# Autodesk Inventor assembly: Tele
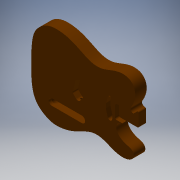
[picture p0: Inventor's stored thumbnail of the model, 180x180]
Saved by Autodesk Inventor 2018 (Build 220112000, 112)
## iProperties
Created: 2021-03-24
Part Number: Tele
Document SubType Name: Assembly
Designer: Charles.Rymal
Author: Charles.Rymal
## Documents named in this file (4)
- C:\Users\Charles.Rymal\source\guitar\CAD\Tele.iam
- C:\Users\Charles.Rymal\source\guitar\CAD\Body.ipt
- C:\Users\Charles.Rymal\source\guitar\CAD\Arduino Spacer.ipt
- C:\Users\Charles.Rymal\source\guitar\CAD\Arduino Due.ipt
## Components (6 placed, 3 different names)
1. Body:1 — Mate:1, Mate:2, Mate:3, Mate:4, Mate:5, Mate:6, Mate:7, Mate:8
2. Arduino Spacer:1 — Mate:4, Mate:6, Mate:10
3. Arduino Spacer:2 — Mate:3, Mate:7
4. Arduino Spacer:3 — Mate:2, Mate:5
5. Arduino Spacer:4 — Mate:1, Mate:8, Mate:9, Mate:11
6. Arduino Due:1 — Mate:9, Mate:10, Mate:11
## Relationships (11: Mate 11)
- Mate:1: Body:1 ↔ Arduino Spacer:4
- Mate:2: Body:1 ↔ Arduino Spacer:3
- Mate:3: Body:1 ↔ Arduino Spacer:2
- Mate:4: Body:1 ↔ Arduino Spacer:1
- Mate:5: Body:1 ↔ Arduino Spacer:3
- Mate:6: Body:1 ↔ Arduino Spacer:1
- Mate:7: Body:1 ↔ Arduino Spacer:2
- Mate:8: Body:1 ↔ Arduino Spacer:4
- Mate:9: Arduino Spacer:4 ↔ Arduino Due:1
- Mate:10: Arduino Spacer:1 ↔ Arduino Due:1
- Mate:11: Arduino Spacer:4 ↔ Arduino Due:1
